# Autodesk Inventor assembly: Climber
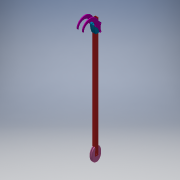
[picture p0: Inventor's stored thumbnail of the model, 180x180]
Saved by Autodesk Inventor 2017 SP1 (Build 210196100, 196)
## iProperties
Created: 2018-03-18
Part Number: Climber
Document SubType Name: Assembly
Designer: Ben
Mass: 328.526 g
Surface Area: 2270.99 cm^2
Volume: 259.198 cm^3
Density: 1.26747 g/cm^3
Author: Ben
## Documents named in this file (5)
- C:\Users\Ben\Desktop\Projects\2018 Robot\Cube Lift\Climber.iam
- C:\Users\Ben\Desktop\Projects\2018 Robot\Cube Lift\climb bar.ipt
- C:\Users\Ben\Desktop\Projects\2018 Robot\Cube Lift\climb slider.ipt
- C:\Users\Ben\Desktop\Projects\2018 Robot\Cube Lift\climb hook.ipt
- C:\Users\Ben\Desktop\Projects\2018 Robot\Cube Lift\climb pulley.ipt
## Components (5 placed, 4 different names)
1. climb bar:1 — Flush:1, Flush:2, Flush:3, Flush:4, Mate:1, Mate:2, Mate:3, Mate:4
2. climb slider:1 — Flush:1, Flush:2, Insert:1, Insert:2, Insert:3, Insert:4
3. climb hook:1 — Insert:1, Insert:2
4. climb hook:2 — Insert:3, Insert:4
5. climb pulley:1 — Mate:2, Mate:3, Mate:4
## Relationships (12: Flush 4, Insert 4, Mate 4)
- Flush:1: climb bar:1 ↔ climb slider:1
- Flush:2: climb bar:1 ↔ climb slider:1
- Insert:1: climb slider:1 ↔ climb hook:1
- Insert:2: climb slider:1 ↔ climb hook:1
- Insert:3: climb slider:1 ↔ climb hook:2
- Insert:4: climb slider:1 ↔ climb hook:2
- Flush:3: climb bar:1
- Flush:4: climb bar:1
- Mate:1: climb bar:1
- Mate:2: climb bar:1 ↔ climb pulley:1
- Mate:3: climb bar:1 ↔ climb pulley:1
- Mate:4: climb bar:1 ↔ climb pulley:1
